# Autodesk Inventor assembly: motor
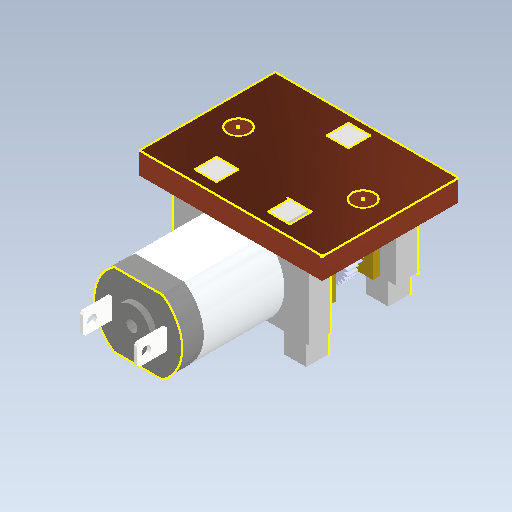
[picture p0: Inventor's stored thumbnail of the model, 512x512]
Saved by Autodesk Inventor 2023 (Build 270158000, 158)
## iProperties
Created: 2023-05-16
Part Number: motor
Document SubType Name: Assembly
Designer: Johnny Jou
Author: Johnny Jou
## Documents named in this file (5)
- C:\Users\Johnny Jou\Documents\GitHub\Areo_Rider_Cabin\car\motor.iam
- C:\Users\Johnny Jou\Documents\GitHub\Areo_Rider_Cabin\car\垃圾\motorbase_1.ipt
- C:\Users\Johnny Jou\Documents\GitHub\Areo_Rider_Cabin\car\垃圾\motorbase_2.ipt
- C:\Users\Johnny Jou\Documents\GitHub\Areo_Rider_Cabin\car\垃圾\motorbase_3.ipt
- C:\Users\Johnny Jou\Documents\GitHub\Areo_Rider_Cabin\car\外抓檔\GA12-N20 Motor-Complet.iam
## Components (5 placed, 4 different names)
1. motorbase_1:1 — 齊平:3, 貼合:1, 貼合:2
2. motorbase_2:1 — 貼合:3, 齊平:4, 貼合:5, 貼合:8
3. motorbase_3:1 — 齊平:3, 貼合:1, 貼合:2, 齊平:4, 齊平:5, 貼合:5, 貼合:6, 貼合:7, 貼合:8
4. motorbase_2:2 — 貼合:4, 齊平:5, 貼合:6, 貼合:9
5. GA12-N20 Motor-Complet:1 [sub-assembly] — 貼合:3, 貼合:4, 貼合:7, 貼合:9
## Relationships (12: Mate 9, Flush 3)
- 齊平:3 [Flush]: motorbase_1:1 ↔ motorbase_3:1
- 貼合:1 [Mate]: motorbase_1:1 ↔ motorbase_3:1
- 貼合:2 [Mate]: motorbase_1:1 ↔ motorbase_3:1
- 貼合:3 [Mate]: motorbase_2:1 ↔ GA12-N20 Motor-Complet:1
- 貼合:4 [Mate]: motorbase_2:2 ↔ GA12-N20 Motor-Complet:1
- 齊平:4 [Flush]: motorbase_2:1 ↔ motorbase_3:1
- 齊平:5 [Flush]: motorbase_3:1 ↔ motorbase_2:2
- 貼合:5 [Mate]: motorbase_2:1 ↔ motorbase_3:1
- 貼合:6 [Mate]: motorbase_3:1 ↔ motorbase_2:2
- 貼合:7 [Mate]: motorbase_3:1 ↔ GA12-N20 Motor-Complet:1
- 貼合:8 [Mate]: motorbase_2:1 ↔ motorbase_3:1
- 貼合:9 [Mate]: motorbase_2:2 ↔ GA12-N20 Motor-Complet:1
